# Autodesk Inventor assembly: leg_upper_left
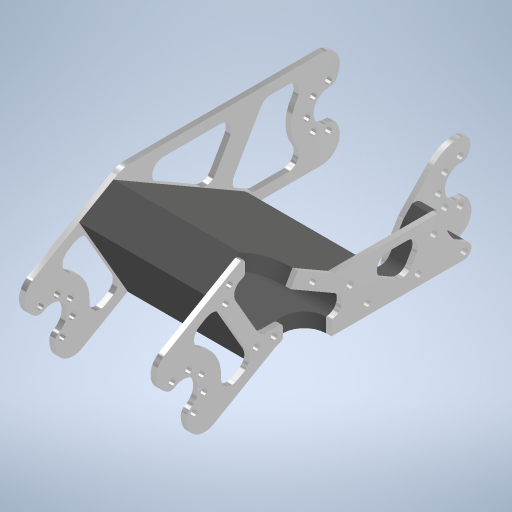
[picture p0: Inventor's stored thumbnail of the model, 512x512]
Saved by Autodesk Inventor 2024.1 (Build 281209000, 209)
## iProperties
Created: 2024-10-11
Part Number: leg_upper_left
Document SubType Name: Assembly
Designer: hibik
Author: hibik
## Documents named in this file (6)
- C:\Users\hibik\Documents\Robomech\HR\Eglantyne\hard\leg\leg_upper_left.iam
- C:\Users\hibik\Documents\Robomech\HR\Eglantyne\hard\leg\leg_upper_outside.ipt
- C:\Users\hibik\Documents\Robomech\HR\Eglantyne\hard\leg\leg_upper_middle_left.ipt
- C:\Users\hibik\Documents\Robomech\HR\Eglantyne\hard\leg\leg_upper_inside_down.ipt
- C:\Users\hibik\Documents\Robomech\HR\Eglantyne\hard\leg\leg_upper_inside_up.ipt
- C:\Users\hibik\Documents\Robomech\HR\Eglantyne\hard\leg\leg_upper_inside_up_base.ipt
## Components (5 placed, 5 different names)
1. leg_upper_outside:1 — 挿入:1, フラッシュ:1
2. leg_upper_middle_left:1 — 挿入:1, フラッシュ:1, 挿入:2, 挿入:3, 挿入:4, 挿入:5, 挿入:6, 挿入:7
3. leg_upper_inside_down:1 — 挿入:2, 挿入:3
4. leg_upper_inside_up:1 — 挿入:4, 挿入:5
5. leg_upper_inside_up_base:1 — 挿入:6, 挿入:7
## Relationships (8: Insert 7, Flush 1)
- 挿入:1 [Insert]: leg_upper_outside:1 ↔ leg_upper_middle_left:1
- フラッシュ:1 [Flush]: leg_upper_outside:1 ↔ leg_upper_middle_left:1
- 挿入:2 [Insert]: leg_upper_middle_left:1 ↔ leg_upper_inside_down:1
- 挿入:3 [Insert]: leg_upper_middle_left:1 ↔ leg_upper_inside_down:1
- 挿入:4 [Insert]: leg_upper_middle_left:1 ↔ leg_upper_inside_up:1
- 挿入:5 [Insert]: leg_upper_middle_left:1 ↔ leg_upper_inside_up:1
- 挿入:6 [Insert]: leg_upper_middle_left:1 ↔ leg_upper_inside_up_base:1
- 挿入:7 [Insert]: leg_upper_middle_left:1 ↔ leg_upper_inside_up_base:1
